# Autodesk Inventor assembly: caster_wheel_2_long
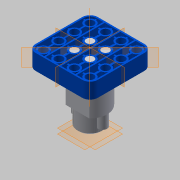
[picture p0: Inventor's stored thumbnail of the model, 180x180]
Saved by Autodesk Inventor 2019.3 (Build 233278000, 278)
## iProperties
Created: 2019-02-11
Part Number: caster_wheel_2_long
Description: STEP AP214
Document SubType Name: Assembly
Designer: Varga Daniel
Sending System: SolidWorks 2018
Preprocessor: SwSTEP 2.0
Title: caster_wheel.STEP
Revision Number: ANY
## Documents named in this file (6)
- C:\!_Dani\!_cloud\OneDrive\!_munka\Revolution\RevvyDemoKit\Structural parts\Demo parts\Caster wheel\Inventor imported\caster_wheel_2\caster_wheel_2_long.iam
- C:\!_Dani\!_cloud\OneDrive\!_munka\Revolution\RevvyDemoKit\Structural parts\Demo parts\Caster wheel\Inventor imported\caster_wheel_base.ipt
- C:\!_Dani\!_cloud\OneDrive\!_munka\Revolution\RevvyDemoKit\Structural parts\Demo parts\Caster wheel\Inventor imported\mini_3pi_caster_wheel.iam
- C:\!_Dani\!_cloud\OneDrive\!_munka\Revolution\RevvyDemoKit\Structural parts\Demo parts\Caster wheel\Inventor imported\Caster_wheel_inner_plug_2.ipt
- C:\!_Dani\!_cloud\OneDrive\!_munka\Revolution\RevvyDemoKit\Structural parts\Demo parts\Caster wheel\Inventor imported\caster_wheel_2.iam
- C:\!_Dani\!_cloud\OneDrive\!_munka\Revolution\RevvyDemoKit\Structural parts\Demo parts\Caster wheel\Inventor imported\Caster_wheel_inner_plug_2\Caster_wheel_inner_plug_2_02.ipt
## Components (3 placed, 3 different names)
1. caster_wheel_base:1 — Mate:2, Flush:1, Mate:3, Mate:4, Mate:5
2. mini_3pi_caster_wheel:1 [sub-assembly] — Angle:1, Tangent:1, Mate:2, Flush:1, Mate:6
3. Caster_wheel_inner_plug_2_02:1 — Mate:3, Mate:4, Mate:5, Mate:6
## Relationships (8: Mate 5, Angle 1, Tangent 1, Flush 1)
- Angle:1 (0 deg): mini_3pi_caster_wheel:1
- Tangent:1: mini_3pi_caster_wheel:1
- Mate:2: caster_wheel_base:1 ↔ mini_3pi_caster_wheel:1
- Flush:1: caster_wheel_base:1 ↔ mini_3pi_caster_wheel:1
- Mate:3: caster_wheel_base:1 ↔ Caster_wheel_inner_plug_2_02:1
- Mate:4: caster_wheel_base:1 ↔ Caster_wheel_inner_plug_2_02:1
- Mate:5: caster_wheel_base:1 ↔ Caster_wheel_inner_plug_2_02:1
- Mate:6: mini_3pi_caster_wheel:1 ↔ Caster_wheel_inner_plug_2_02:1
